# Autodesk Inventor assembly: s-assy-ring_gear-2
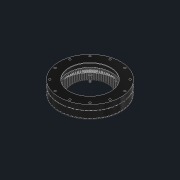
[picture p0: Inventor's stored thumbnail of the model, 180x180]
Saved by Autodesk Inventor 2022 (Build 260153000, 153)
## iProperties
Created: 2021-07-12
Part Number: s-assy-ring_gear-2
Document SubType Name: Assembly
Designer: yuta0
Mass: 180.782 g
Surface Area: 832.349 cm^2
Volume: 122.833 cm^3
Density: 1.47176 g/cm^3
Author: yuta0
## Documents named in this file (8)
- C:\Users\yuta0\Documents\GitHub\catchrobo_hardware\assy-robot\s-assy-ring_gear-2.iam
- C:\Users\yuta0\Documents\GitHub\catchrobo_hardware\assy-robot\base33.ipt
- C:\Users\yuta0\Documents\GitHub\catchrobo_hardware\assy-robot\carbon_plate13.ipt
- C:\Users\yuta0\Documents\GitHub\catchrobo_hardware\assy-robot\carbon_plate9.ipt
- C:\Users\yuta0\Documents\GitHub\catchrobo_hardware\assy-robot\LBNR2.ipt
- C:\Users\yuta0\Documents\GitHub\catchrobo_hardware\assy-robot\CBSTSR4-14.ipt
- C:\Users\yuta0\Documents\GitHub\catchrobo_hardware\assy-scara\scara-base3.ipt
- C:\Users\yuta0\Documents\GitHub\catchrobo_hardware\assy-robot\s-assy-ring_gear.iam
## Components (9 placed, 6 different names)
1. base33:1 — フラッシュ:2, メイト:5, メイト:6, メイト:11, メイト:41, メイト:52
2. scara-base3:1 — メイト:11, メイト:12, メイト:31
3. carbon_plate13:1 — メイト:4, メイト:5, メイト:6, メイト:12
4. carbon_plate9:1 — メイト:32, メイト:41, メイト:48, メイト:49, メイト:50, メイト:52
5. LBNR2:1 — メイト:48
6. CBSTSR4-14:1 — メイト:49, メイト:50
7. CBSTSR4-14:2
8. CBSTSR4-14:3
9. CBSTSR4-14:4
## Component patterns: (4 elements, first: CBSTSR4-14:1)
## Relationships (13: Mate 12, Flush 1)
- フラッシュ:2 [Flush]: base33:1
- メイト:4 [Mate]: carbon_plate13:1
- メイト:5 [Mate]: base33:1 ↔ carbon_plate13:1
- メイト:6 [Mate]: base33:1 ↔ carbon_plate13:1
- メイト:11 [Mate]: base33:1 ↔ scara-base3:1
- メイト:12 [Mate]: scara-base3:1 ↔ carbon_plate13:1
- メイト:31 [Mate]: scara-base3:1
- メイト:32 [Mate]: carbon_plate9:1
- メイト:41 [Mate]: base33:1 ↔ carbon_plate9:1
- メイト:48 [Mate]: carbon_plate9:1 ↔ LBNR2:1
- メイト:49 [Mate]: carbon_plate9:1 ↔ CBSTSR4-14:1
- メイト:50 [Mate]: carbon_plate9:1 ↔ CBSTSR4-14:1
- メイト:52 [Mate]: base33:1 ↔ carbon_plate9:1
